# Autodesk Inventor assembly: ServoWithShaftAssembly
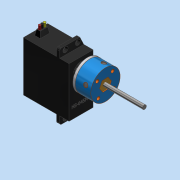
[picture p0: Inventor's stored thumbnail of the model, 180x180]
Saved by Autodesk Inventor 2017.3 (Build 213256000, 256)
## iProperties
Created: 2016-11-03
Part Number: ServoWithShaftAssembly
Document SubType Name: Assembly
Designer: techn
Mass: 47.1861 g
Surface Area: 102.032 cm^2
Volume: 34.7603 cm^3
Density: 1.35747 g/cm^3
Author: techn
## Documents named in this file (8)
- G:\Projects\Submarine\Submarine-project\CAD\common\3mmShaftToServo\ServoWithShaftAssembly.iam
- G:\Projects\Submarine\Submarine-project\CAD\common\HitecServo\HitecServoAssembly.iam
- G:\Projects\Submarine\Submarine-project\CAD\common\3mmShaftToServo\.125InchServoDrivenShaft.ipt
- G:\Projects\Submarine\Submarine-project\CAD\common\3mmShaftToServo\HexNutShaftServoCoupler.ipt
- G:\Projects\Submarine\Submarine-project\CAD\common\3mmShaftToServo\.125InchShaftHexNut.ipt
- G:\Projects\Submarine\Submarine-project\CAD\common\HitecServo\ServoHornDisc.ipt
- G:\Projects\Submarine\Submarine-project\CAD\common\screws\ScrewPlastic_4_20_.5inch.ipt
- G:\Projects\Submarine\Submarine-project\CAD\aft\encoder\EncoderMagnet.ipt
## Components (13 placed, 7 different names)
1. HitecServoAssembly:1 [sub-assembly] — Mate:1, Mate:2
2. .125InchServoDrivenShaft:1 — Mate:3, Mate:5, Flush:1
3. HexNutShaftServoCoupler:1 — Mate:3, Mate:6, Mate:7, Mate:8, Mate:9, Angle:1, Mate:12, Mate:13
4. .125InchShaftHexNut:1 — Mate:5, Mate:6, Angle:1, Flush:1
5. ServoHornDisc:1 — Mate:1, Mate:2, Mate:7, Mate:8, Mate:9, Mate:10, Mate:11
6. ScrewPlastic_4_20_.5inch:1 — Mate:10, Mate:11
7. ScrewPlastic_4_20_.5inch:2
8. ScrewPlastic_4_20_.5inch:3
9. ScrewPlastic_4_20_.5inch:4
10. EncoderMagnet:1 — Mate:12, Mate:13
11. EncoderMagnet:2
12. EncoderMagnet:3
13. EncoderMagnet:4
## Component patterns: (4 elements, first: ScrewPlastic_4_20_.5inch:1), (4 elements, first: EncoderMagnet:1)
## Relationships (14: Mate 12, Angle 1, Flush 1)
- Mate:1: HitecServoAssembly:1 ↔ ServoHornDisc:1
- Mate:2: HitecServoAssembly:1 ↔ ServoHornDisc:1
- Mate:3: .125InchServoDrivenShaft:1 ↔ HexNutShaftServoCoupler:1
- Mate:5: .125InchServoDrivenShaft:1 ↔ .125InchShaftHexNut:1
- Mate:6: HexNutShaftServoCoupler:1 ↔ .125InchShaftHexNut:1
- Mate:7: HexNutShaftServoCoupler:1 ↔ ServoHornDisc:1
- Mate:8: HexNutShaftServoCoupler:1 ↔ ServoHornDisc:1
- Mate:9: HexNutShaftServoCoupler:1 ↔ ServoHornDisc:1
- Angle:1 (0 deg): HexNutShaftServoCoupler:1 ↔ .125InchShaftHexNut:1
- Flush:1: .125InchServoDrivenShaft:1 ↔ .125InchShaftHexNut:1
- Mate:10: ServoHornDisc:1 ↔ ScrewPlastic_4_20_.5inch:1
- Mate:11: ServoHornDisc:1 ↔ ScrewPlastic_4_20_.5inch:1
- Mate:12: HexNutShaftServoCoupler:1 ↔ EncoderMagnet:1
- Mate:13: HexNutShaftServoCoupler:1 ↔ EncoderMagnet:1
